# Autodesk Inventor assembly: Assembly1
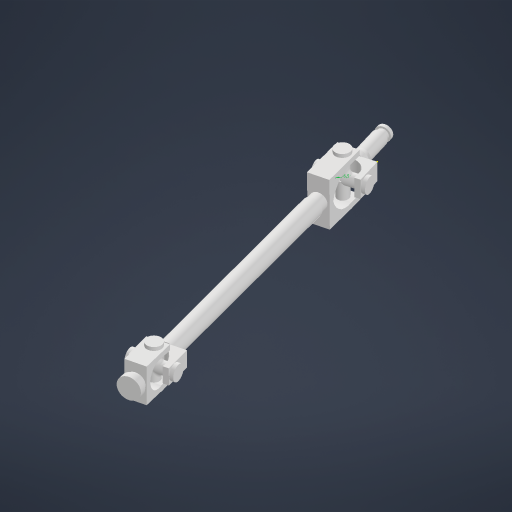
[picture p0: Inventor's stored thumbnail of the model, 512x512]
Saved by Autodesk Inventor 2023 (Build 270158030, 158C)
## iProperties
Created: 2023-03-29
Part Number: Assembly1
Document SubType Name: Assembly
Designer: Monster
Author: Monster
## Documents named in this file (9)
- C:\Users\Monster\Desktop\Ders\UKA\shaft toplam\shaft3\Assembly1.iam
- C:\Users\Monster\Desktop\Ders\UKA\shaft toplam\shaft3\Part3.1.ipt
- C:\Users\Monster\Desktop\Ders\UKA\shaft toplam\shaft3\shaft 4 kol.ipt
- C:\Users\Monster\Desktop\Ders\UKA\shaft toplam\shaft3\vida3.1.ipt
- C:\Users\Monster\Desktop\Ders\UKA\shaft toplam\shaft3\Part3.4.ipt
- C:\Users\Monster\Desktop\Ders\UKA\shaft toplam\shaft3\Part3.5.ipt
- C:\Users\Monster\Desktop\Ders\UKA\shaft toplam\shaft3\shaft 4 kol büyük kısım.ipt
- C:\Users\Monster\Desktop\Ders\UKA\shaft toplam\shaft3\vida3.1(uzun).ipt
- C:\Users\Monster\Desktop\Ders\UKA\shaft toplam\shaft3\vida3.2(kısa).ipt
## Components (13 placed, 8 different names)
1. Part3.1:1 — Mate:12, Mate:27, Mate:28, Mate:34
2. Part3.4:1 — Mate:29, Mate:39
3. shaft 4 kol:2 — Mate:12, Mate:15, Mate:17, Mate:19, Mate:20, Mate:21, Mate:23, Mate:24, Mate:25, Mate:26
4. vida3.1:6 — Mate:15, Mate:20
5. vida3.1:7 — Mate:17, Mate:21, Mate:22
6. Part3.5:1 — Mate:19, Mate:22
7. vida3.1:8 — Mate:23, Mate:24
8. vida3.1:9 — Mate:25, Mate:26, Mate:27
9. shaft 4 kol büyük kısım:1 — Mate:28, Mate:29, Mate:30, Mate:31, Mate:32, Mate:33, Mate:35, Mate:36, Mate:37, Mate:38
10. vida3.1(uzun):1 — Mate:32, Mate:33
11. vida3.1(uzun):2 — Mate:30, Mate:31, Mate:34
12. vida3.2(kısa):1 — Mate:35, Mate:36
13. vida3.2(kısa):2 — Mate:37, Mate:38, Mate:39
## Relationships (24: Mate 24)
- Mate:12: Part3.1:1 ↔ shaft 4 kol:2
- Mate:15: shaft 4 kol:2 ↔ vida3.1:6
- Mate:17: shaft 4 kol:2 ↔ vida3.1:7
- Mate:19: shaft 4 kol:2 ↔ Part3.5:1
- Mate:20: shaft 4 kol:2 ↔ vida3.1:6
- Mate:21: shaft 4 kol:2 ↔ vida3.1:7
- Mate:22: vida3.1:7 ↔ Part3.5:1
- Mate:23: shaft 4 kol:2 ↔ vida3.1:8
- Mate:24: shaft 4 kol:2 ↔ vida3.1:8
- Mate:25: shaft 4 kol:2 ↔ vida3.1:9
- Mate:26: shaft 4 kol:2 ↔ vida3.1:9
- Mate:27: Part3.1:1 ↔ vida3.1:9
- Mate:28: Part3.1:1 ↔ shaft 4 kol büyük kısım:1
- Mate:29: Part3.4:1 ↔ shaft 4 kol büyük kısım:1
- Mate:30: shaft 4 kol büyük kısım:1 ↔ vida3.1(uzun):2
- Mate:31: shaft 4 kol büyük kısım:1 ↔ vida3.1(uzun):2
- Mate:32: shaft 4 kol büyük kısım:1 ↔ vida3.1(uzun):1
- Mate:33: shaft 4 kol büyük kısım:1 ↔ vida3.1(uzun):1
- Mate:34: Part3.1:1 ↔ vida3.1(uzun):2
- Mate:35: shaft 4 kol büyük kısım:1 ↔ vida3.2(kısa):1
- Mate:36: shaft 4 kol büyük kısım:1 ↔ vida3.2(kısa):1
- Mate:37: shaft 4 kol büyük kısım:1 ↔ vida3.2(kısa):2
- Mate:38: shaft 4 kol büyük kısım:1 ↔ vida3.2(kısa):2
- Mate:39: Part3.4:1 ↔ vida3.2(kısa):2
